# Autodesk Inventor assembly: MA
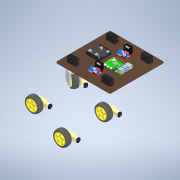
[picture p0: Inventor's stored thumbnail of the model, 180x180]
Saved by Autodesk Inventor 2022.3 (Build 263350000, 350)
## iProperties
Created: 2022-04-28
Part Number: MA
Document SubType Name: Assembly
Designer: Robert Nies
Author: Robert Nies
## Documents named in this file (10)
- C:\Users\rober\PycharmProjects\SwervoDrive\CAD\MA.iam
- C:\Users\rober\PycharmProjects\SwervoDrive\CAD\CAD_Lib\RPi\Raspberry Pi 4 Model B.iam
- C:\Users\rober\PycharmProjects\SwervoDrive\CAD\CAD_Lib\L298N Driver DC Motor, Stepper Motor.ipt
- C:\Users\rober\PycharmProjects\SwervoDrive\CAD\CAD_Lib\Battery\4x AA Alkaline 1.5 V Battery Pack.iam
- C:\Users\rober\PycharmProjects\SwervoDrive\CAD\RobotBase.ipt
- C:\Users\rober\PycharmProjects\SwervoDrive\CAD\CAD_Lib\Servo\Servo Motor MG996R.iam
- C:\Users\rober\PycharmProjects\SwervoDrive\CAD\CAD_Lib\drive_motor.ipt
- C:\Users\rober\PycharmProjects\SwervoDrive\CAD\CAD_Lib\wheel.ipt
- C:\Users\rober\PycharmProjects\SwervoDrive\CAD\CAD_Lib\Servo\attachmentStraight.ipt
- C:\Users\rober\PycharmProjects\SwervoDrive\CAD\CAD_Lib\Servo\SwerveBracket.ipt
## Components (22 placed, 9 different names)
1. Raspberry Pi [sub-assembly] — Mate:1, Flush:1, Flush:2
2. Dual Motor Driver:1 — Mate:4, Flush:5, Flush:6
3. Dual Motor Driver:2 — Mate:3, Flush:5, Flush:7
4. Battery Pack [sub-assembly] — Mate:2, Flush:3, Flush:4
5. RobotBase:1 — Mate:1, Flush:1, Flush:2, Mate:2, Flush:3, Flush:4, Mate:3, Mate:4, Flush:6, Flush:7, Mate:17, Mate:18, Mate:19, Mate:20, Mate:21, Mate:22, Mate:23, Mate:24, Mate:25, Mate:26, Mate:27, Mate:28
6. attachmentStraight:3 — Rotational:2, Rotational:7
7. Servo Motor MG996R:1 [sub-assembly] — Mate:26, Mate:27, Mate:28, Rotational:2
8. wheel:6
9. drive_motor:6 — Rotational:8, Rotational:9
10. SwerveBracket:1 — Rotational:7, Rotational:8, Rotational:9
11. attachmentStraight:4 — Rotational:1
12. drive_motor:5
13. wheel:5
14. Servo Motor MG996R:2 [sub-assembly] — Mate:17, Mate:18, Mate:19, Rotational:1
15. Servo Motor MG996R:3 [sub-assembly] — Mate:23, Mate:24, Mate:25, Rotational:4
16. attachmentStraight:2 — Rotational:4
17. drive_motor:1 — Mate:5, Mate:6, Mate:7
18. wheel:1 — Mate:5, Mate:6, Mate:7
19. Servo Motor MG996R:4 [sub-assembly] — Mate:20, Mate:21, Mate:22, Rotational:3
20. drive_motor:7
21. wheel:7
22. attachmentStraight:1 — Rotational:3
## Relationships (42: Mate 28, Flush 7, RevoluteJoint 7)
- Mate:1: Raspberry Pi ↔ RobotBase:1
- Flush:1 (101.6 mm): Raspberry Pi ↔ RobotBase:1
- Flush:2 (50.8 mm): Raspberry Pi ↔ RobotBase:1
- Mate:2: Battery Pack ↔ RobotBase:1
- Flush:3 (101.6 mm): Battery Pack ↔ RobotBase:1
- Flush:4 (38.1 mm): Battery Pack ↔ RobotBase:1
- Mate:3: Dual Motor Driver:2 ↔ RobotBase:1
- Mate:4: Dual Motor Driver:1 ↔ RobotBase:1
- Flush:5: Dual Motor Driver:1 ↔ Dual Motor Driver:2
- Flush:6 (38.1 mm): Dual Motor Driver:1 ↔ RobotBase:1
- Flush:7 (38.1 mm): Dual Motor Driver:2 ↔ RobotBase:1
- Mate:5: drive_motor:1 ↔ wheel:1
- Mate:6: drive_motor:1 ↔ wheel:1
- Mate:7: drive_motor:1 ↔ wheel:1
- [Mate]: drive_motor:5 ↔ wheel:5
- [Mate]: drive_motor:5 ↔ wheel:5
- [Mate]: drive_motor:5 ↔ wheel:5
- [Mate]: wheel:6 ↔ drive_motor:6
- [Mate] (2.54 mm): wheel:6 ↔ drive_motor:6
- [Mate]: wheel:6 ↔ drive_motor:6
- [Mate]: drive_motor:7 ↔ wheel:7
- [Mate]: drive_motor:7 ↔ wheel:7
- [Mate]: drive_motor:7 ↔ wheel:7
- Mate:17: RobotBase:1 ↔ Servo Motor MG996R:2
- Mate:18: RobotBase:1 ↔ Servo Motor MG996R:2
- Mate:19: RobotBase:1 ↔ Servo Motor MG996R:2
- Mate:20: RobotBase:1 ↔ Servo Motor MG996R:4
- Mate:21: RobotBase:1 ↔ Servo Motor MG996R:4
- Mate:22: RobotBase:1 ↔ Servo Motor MG996R:4
- Mate:23: RobotBase:1 ↔ Servo Motor MG996R:3
- Mate:24: RobotBase:1 ↔ Servo Motor MG996R:3
- Mate:25: RobotBase:1 ↔ Servo Motor MG996R:3
- Mate:26: RobotBase:1 ↔ Servo Motor MG996R:1
- Mate:27: RobotBase:1 ↔ Servo Motor MG996R:1
- Mate:28: RobotBase:1 ↔ Servo Motor MG996R:1
- Rotational:1 [RevoluteJoint]: attachmentStraight:4 ↔ Servo Motor MG996R:2
- Rotational:2 [RevoluteJoint]: attachmentStraight:3 ↔ Servo Motor MG996R:1
- Rotational:3 [RevoluteJoint]: Servo Motor MG996R:4 ↔ attachmentStraight:1
- Rotational:4 [RevoluteJoint]: Servo Motor MG996R:3 ↔ attachmentStraight:2
- Rotational:7 [RevoluteJoint]: attachmentStraight:3 ↔ SwerveBracket:1
- Rotational:8 [RevoluteJoint]: drive_motor:6 ↔ SwerveBracket:1
- Rotational:9 [RevoluteJoint]: drive_motor:6 ↔ SwerveBracket:1
## Named parameters: d14_d11 = 0 mm, d15_d12 = 0 mm, d16_d13 = 0 mm, d17_d14_d11 = 0 mm, d18_d15_d12 = 2.54 mm, d19_d16_d13 = 0 mm, d20_d14_d11 = 0 mm, d21_d15_d12 = 0 mm, d22_d16_d13 = 0 mm
